# Autodesk Inventor assembly: Carriage_Assembly
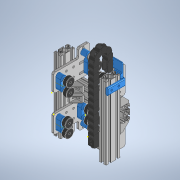
[picture p0: Inventor's stored thumbnail of the model, 180x180]
Saved by Autodesk Inventor 2021 (Build 250183000, 183)
## iProperties
Created: 2021-09-08
Part Number: Carriage_Assembly
Document SubType Name: Assembly
Designer: Jorian Brusind
Author: Jorian Brusind
## Documents named in this file (10)
- C:\Users\Jorian Brusind\Documents\GitHub\PersonalProjects\HyperRail\Inventor Files\Carriage_Assembly.iam
- C:\Users\Jorian Brusind\Documents\GitHub\PersonalProjects\Inventor Projects\Useful models\8020_Sets\IPT_20_Series\IPT_20_Series\20-2040_200mm.ipt
- C:\Users\Jorian Brusind\Documents\GitHub\PersonalProjects\Inventor Projects\Useful models\8020_Sets\IPT_20_Series\IPT_20_Series\20-2040_150mm.ipt
- C:\Users\Jorian Brusind\Documents\GitHub\PersonalProjects\HyperRail\Inventor Files\X_CarriageL_V2_0_Short.iam
- C:\Users\Jorian Brusind\Documents\GitHub\PersonalProjects\HyperRail\Inventor Files\X_CarriageR_V2_0_Short.iam
- C:\Users\Jorian Brusind\Documents\GitHub\PersonalProjects\HyperRail\Inventor Files\X_CarriageR_V2_0.iam
- C:\Users\Jorian Brusind\Documents\GitHub\PersonalProjects\HyperRail\Inventor Files\X_Carriage_V2_0.iam
- C:\Users\Jorian Brusind\Documents\GitHub\PersonalProjects\HyperRail\Inventor Files\Cable_Guide_End.ipt
- C:\Users\Jorian Brusind\Documents\GitHub\PersonalProjects\HyperRail\Inventor Files\17mmBeltGuide.ipt
- C:\Users\Jorian Brusind\Documents\GitHub\PersonalProjects\Inventor Projects\Useful models\8020_Sets\IPT_20_Series\Extra_20_Series\8020_14056m\14056_m.ipt
## Components (15 placed, 9 different names)
1. 20-2040_200mm:1 — Mate:1, Flush:1, Mate:2, Flush:2, Mate:3, Mate:4, Mate:5, Mate:6, Mate:7, Flush:3, Mate:9, Flush:6, Flush:7, Flush:11, Flush:12, Mate:24, Mate:25, Mate:29
2. 20-2040_200mm:2 — Mate:10, Mate:11, Flush:4, Flush:5, Mate:12, Mate:13, Flush:6, Flush:7, Mate:15, Flush:8, Mate:16, Mate:17, Mate:18, Mate:19, Flush:9, Flush:10
3. 20-2040_150mm:1 — Flush:3, Mate:8, Mate:9, Mate:20, Mate:21, Mate:22, Mate:23, Mate:26, Flush:14, Mate:27, Flush:15
4. X_CarriageL_V2_0_Short:1 [sub-assembly] — Mate:10, Flush:5, Mate:13, Mate:14
5. X_CarriageR_V2_0_Short:1 [sub-assembly] — Mate:11, Flush:4, Mate:12, Mate:30
6. X_CarriageR_V2_0:1 [sub-assembly] — Mate:1, Flush:1, Mate:2, Mate:8, Mate:14
7. X_Carriage_V2_0:1 [sub-assembly] — Flush:2, Mate:3, Mate:4
8. Cable_Guide_End:1 — Mate:15, Flush:8, Mate:16
9. 17mmBeltGuide:1 — Mate:17, Mate:30
10. 14056_m:1 — Mate:19, Mate:21, Flush:9
11. 14056_m:2 — Mate:18, Mate:20, Flush:10
12. 14056_m:3 — Mate:22, Flush:12, Flush:13
13. 14056_m:4 — Mate:23, Flush:11, Flush:13, Mate:24
14. 14056_m:5 — Mate:27, Mate:29, Flush:15
15. 14056_m:6 — Mate:25, Mate:26, Flush:14
## Relationships (44: Mate 29, Flush 15)
- Mate:1: 20-2040_200mm:1 ↔ X_CarriageR_V2_0:1
- Flush:1: 20-2040_200mm:1 ↔ X_CarriageR_V2_0:1
- Mate:2 (5 mm): 20-2040_200mm:1 ↔ X_CarriageR_V2_0:1
- Flush:2: 20-2040_200mm:1 ↔ X_Carriage_V2_0:1
- Mate:3: 20-2040_200mm:1 ↔ X_Carriage_V2_0:1
- Mate:4 (5 mm): 20-2040_200mm:1 ↔ X_Carriage_V2_0:1
- Mate:5: 20-2040_200mm:1
- Mate:6: 20-2040_200mm:1
- Mate:7: 20-2040_200mm:1
- Flush:3: 20-2040_200mm:1 ↔ 20-2040_150mm:1
- Mate:8 (5 mm): 20-2040_150mm:1 ↔ X_CarriageR_V2_0:1
- Mate:9 (3 mm): 20-2040_200mm:1 ↔ 20-2040_150mm:1
- Mate:10: 20-2040_200mm:2 ↔ X_CarriageL_V2_0_Short:1
- Mate:11: 20-2040_200mm:2 ↔ X_CarriageR_V2_0_Short:1
- Flush:4: 20-2040_200mm:2 ↔ X_CarriageR_V2_0_Short:1
- Flush:5: 20-2040_200mm:2 ↔ X_CarriageL_V2_0_Short:1
- Mate:12 (3 mm): 20-2040_200mm:2 ↔ X_CarriageR_V2_0_Short:1
- Mate:13 (3 mm): 20-2040_200mm:2 ↔ X_CarriageL_V2_0_Short:1
- Flush:6: 20-2040_200mm:1 ↔ 20-2040_200mm:2
- Flush:7: 20-2040_200mm:1 ↔ 20-2040_200mm:2
- Mate:14 (30 mm): X_CarriageL_V2_0_Short:1 ↔ X_CarriageR_V2_0:1
- Mate:15: 20-2040_200mm:2 ↔ Cable_Guide_End:1
- Flush:8: 20-2040_200mm:2 ↔ Cable_Guide_End:1
- Mate:16: 20-2040_200mm:2 ↔ Cable_Guide_End:1
- Mate:17: 20-2040_200mm:2 ↔ 17mmBeltGuide:1
- Mate:18: 20-2040_200mm:2 ↔ 14056_m:2
- Mate:19: 20-2040_200mm:2 ↔ 14056_m:1
- Mate:20: 20-2040_150mm:1 ↔ 14056_m:2
- Mate:21: 20-2040_150mm:1 ↔ 14056_m:1
- Flush:9: 20-2040_200mm:2 ↔ 14056_m:1
- Flush:10: 20-2040_200mm:2 ↔ 14056_m:2
- Mate:22: 20-2040_150mm:1 ↔ 14056_m:3
- Mate:23: 20-2040_150mm:1 ↔ 14056_m:4
- Flush:11: 20-2040_200mm:1 ↔ 14056_m:4
- Flush:12: 20-2040_200mm:1 ↔ 14056_m:3
- Flush:13: 14056_m:3 ↔ 14056_m:4
- Mate:24: 20-2040_200mm:1 ↔ 14056_m:4
- Mate:25: 20-2040_200mm:1 ↔ 14056_m:6
- Mate:26: 20-2040_150mm:1 ↔ 14056_m:6
- Flush:14: 20-2040_150mm:1 ↔ 14056_m:6
- Mate:27: 20-2040_150mm:1 ↔ 14056_m:5
- Mate:29: 20-2040_200mm:1 ↔ 14056_m:5
- Flush:15: 20-2040_150mm:1 ↔ 14056_m:5
- Mate:30: X_CarriageR_V2_0_Short:1 ↔ 17mmBeltGuide:1
